# Autodesk Inventor assembly: Biblow Assssssssemblee
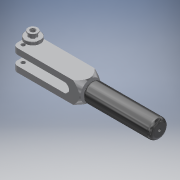
[picture p0: Inventor's stored thumbnail of the model, 180x180]
Saved by Autodesk Inventor 2017.3 (Build 213256000, 256)
## iProperties
Created: 2017-04-21
Part Number: Biblow Assssssssemblee
Document SubType Name: Assembly
Designer: 193515
Author: 193515
## Documents named in this file (10)
- C:\Users\rbibb\Desktop\8.1\Biblow Asemblee.iam
- C:\Users\rbibb\Desktop\8.1\handle bar.ipt
- C:\Users\rbibb\Desktop\8.1\middle handle piece (hard).ipt
- C:\Users\rbibb\Desktop\8.1\Part2.ipt
- C:\Users\rbibb\Desktop\8.1\Roller Inner Bearing.ipt
- C:\Users\rbibb\Desktop\8.1\Roller Outer Bearing.ipt
- C:\Users\rbibb\Desktop\8.1\Roller Spacer.ipt
- C:\Users\rbibb\Desktop\8.1\Roller Inner Bearing_MIR.ipt
- C:\Users\rbibb\Desktop\8.1\Roller Outer Bearing_MIR.ipt
- C:\Users\rbibb\Desktop\8.1\Roller Spacer_MIR.ipt
## Components (9 placed, 9 different names)
1. middle handle piece (hard):1 — Rotational:1, Rigid:2, Flush:1
2. Part2:1 — Rotational:1, Rotational:2
3. handle bar:1 — Rotational:2
4. Roller Inner Bearing:1 — Rotational:3, Rotational:4
5. Roller Outer Bearing:1 — Rigid:2, Rotational:3
6. Roller Spacer:1 — Rotational:4
7. Roller Inner Bearing_MIR:1 — Rotational:5, Rotational:6
8. Roller Outer Bearing_MIR:1 — Rotational:5
9. Roller Spacer_MIR:1 — Rotational:6
## Relationships (8: RevoluteJoint 6, WeldJoint 1, Flush 1)
- Rotational:1 [RevoluteJoint]: middle handle piece (hard):1 ↔ Part2:1
- Rotational:2 [RevoluteJoint]: Part2:1 ↔ handle bar:1
- Rigid:2 [WeldJoint]: middle handle piece (hard):1 ↔ Roller Outer Bearing:1
- Rotational:3 [RevoluteJoint]: Roller Inner Bearing:1 ↔ Roller Outer Bearing:1
- Rotational:4 [RevoluteJoint]: Roller Inner Bearing:1 ↔ Roller Spacer:1
- Flush:1 (7.9375 mm): middle handle piece (hard):1
- Rotational:5 [RevoluteJoint]: Roller Inner Bearing_MIR:1 ↔ Roller Outer Bearing_MIR:1
- Rotational:6 [RevoluteJoint]: Roller Inner Bearing_MIR:1 ↔ Roller Spacer_MIR:1
